# Autodesk Inventor assembly: locking_demo
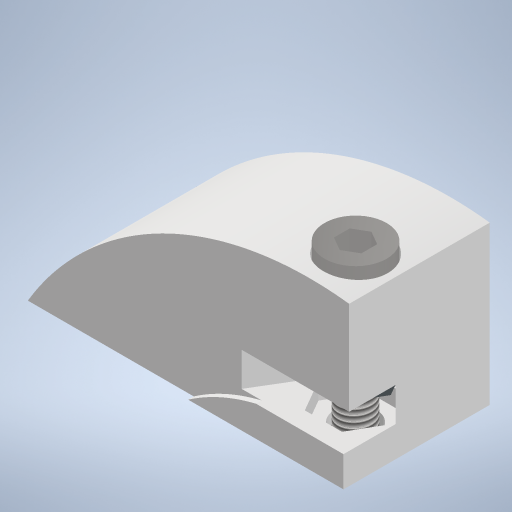
[picture p0: Inventor's stored thumbnail of the model, 512x512]
Saved by Autodesk Inventor 2023 (Build 270158000, 158)
## iProperties
Created: 2023-05-14
Part Number: locking_demo
Document SubType Name: Assembly
Designer: maste
Author: maste
## Documents named in this file (4)
- C:\Users\maste\Documents\GitHub\Remote-Stethoscope\3D_models\ThonkLabs 1ne\SeparateDiaphragm\locking_demo.iam
- C:\Users\maste\Documents\GitHub\Remote-Stethoscope\3D_models\ThonkLabs 1ne\SurfaceContact\PiezoMount.ipt
- C:\Users\maste\Documents\GitHub\Remote-Stethoscope\3D_models\ThonkLabs 1ne\SurfaceContact\fasten_bolt.ipt
- C:\Users\maste\Documents\GitHub\Remote-Stethoscope\3D_models\ThonkLabs 1ne\SurfaceContact\fasten_nut.ipt
## Components (3 placed, 3 different names)
1. PiezoMount:1 — Mate:1, Mate:2, Mate:4
2. fasten_bolt:1 — Mate:3, Mate:4
3. fasten_nut:1 — Mate:1, Mate:2, Mate:3
## Relationships (4: Mate 4)
- Mate:1: PiezoMount:1 ↔ fasten_nut:1
- Mate:2: PiezoMount:1 ↔ fasten_nut:1
- Mate:3: fasten_bolt:1 ↔ fasten_nut:1
- Mate:4: PiezoMount:1 ↔ fasten_bolt:1
